# Autodesk Inventor assembly: drone arm top
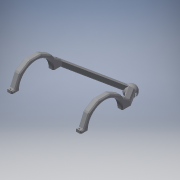
[picture p0: Inventor's stored thumbnail of the model, 180x180]
Saved by Autodesk Inventor 2016 (Build 200138000, 138)
## iProperties
Created: 2018-04-04
Part Number: drone arm top
Document SubType Name: Assembly
Designer: student
Author: student
## Documents named in this file (3)
- C:\Users\student.MVTHS-ENG-S15\Documents\drone\drone arm top.iam
- C:\Users\student.MVTHS-ENG-S15\Documents\drone\Solid1_1.ipt
- C:\Users\student.MVTHS-ENG-S15\Documents\drone\2.ipt
## Components (2 placed, 2 different names)
1. 2:2 — Mate:1, Tangent:1
2. Solid1_1:1 — Mate:1, Tangent:1
## Relationships (2: Mate 1, Tangent 1)
- Mate:1: 2:2 ↔ Solid1_1:1
- Tangent:1: 2:2 ↔ Solid1_1:1
